# Autodesk Inventor assembly: brace
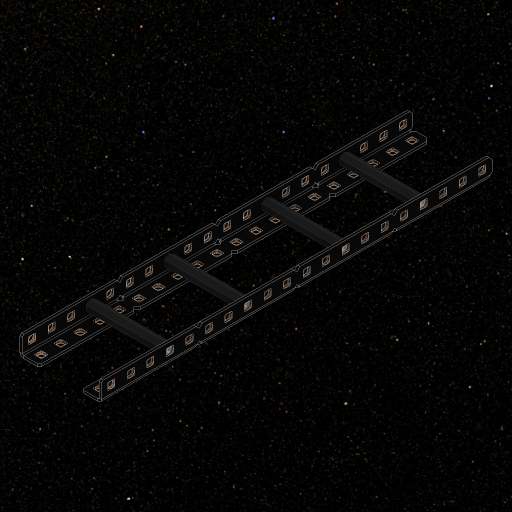
[picture p0: Inventor's stored thumbnail of the model, 512x512]
Saved by Autodesk Inventor 2024 (Build 280153000, 153)
## iProperties
Created: 2024-02-24
Part Number: brace
Document SubType Name: Assembly
Designer: Averey Ku
Author: Averey Ku
## Documents named in this file (5)
- D:\vex_robotics\hardware\cad\lil_zoom\intake\brace.iam
- D:\vex_robotics\hardware\cad\VEX-CAD-Inventor-1.41\Structure\Angle\Aluminum 1x1\Alu Angle 1x1x20.ipt
- D:\vex_robotics\hardware\cad\VEX-CAD-Inventor-1.41\Structure\C Channel\Aluminum 1x2x1\Alu C 1x2x1x4.ipt
- D:\vex_robotics\hardware\cad\VEX-CAD-Inventor-1.41\Structure\Standoff\Standoff 2.00.ipt
- D:\vex_robotics\hardware\cad\VEX-CAD-Inventor-1.41\Structure\Standoff.ipt
## Components (7 placed, 3 different names)
1. Alu Angle 1x1x20:1 — Insert:1, Mate:1, Insert:3, Insert:4
2. Alu Angle 1x1x20:2 — Insert:2, Mate:2, Insert:5, Insert:6
3. Alu C 1x2x1x4:1 — Insert:1, Mate:1, Insert:2, Mate:2
4. Standoff 2.00:1 — Insert:3
5. Standoff 2.00:2 — Insert:4
6. Standoff 2.00:3 — Insert:5
7. Standoff 2.00:4 — Insert:6
## Relationships (8: Insert 6, Mate 2)
- Insert:1: Alu Angle 1x1x20:1 ↔ Alu C 1x2x1x4:1
- Mate:1: Alu Angle 1x1x20:1 ↔ Alu C 1x2x1x4:1
- Insert:2: Alu Angle 1x1x20:2 ↔ Alu C 1x2x1x4:1
- Mate:2: Alu Angle 1x1x20:2 ↔ Alu C 1x2x1x4:1
- Insert:3: Alu Angle 1x1x20:1 ↔ Standoff 2.00:1
- Insert:4: Alu Angle 1x1x20:1 ↔ Standoff 2.00:2
- Insert:5: Alu Angle 1x1x20:2 ↔ Standoff 2.00:3
- Insert:6: Alu Angle 1x1x20:2 ↔ Standoff 2.00:4
